# Autodesk Inventor assembly: GarageAndBracketFlatBracket
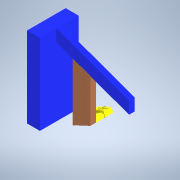
[picture p0: Inventor's stored thumbnail of the model, 180x180]
Saved by Autodesk Inventor 2022.2 (Build 262287000, 287)
## iProperties
Created: 2021-11-26
Part Number: GarageAndBracketFlatBracket
Document SubType Name: Assembly
Designer: robst
Author: robst
## Documents named in this file (4)
- C:\git\CAD-Development\robSteele\ShapeWays\GlobalMeteorNetwork\GarageAndBracketFlatBracket.iam
- C:\git\CAD-Development\robSteele\ShapeWays\GlobalMeteorNetwork\GarageSegment.ipt
- C:\git\CAD-Development\robSteele\ShapeWays\GlobalMeteorNetwork\caseLowerPortionV02.ipt
- C:\git\CAD-Development\robSteele\ShapeWays\GlobalMeteorNetwork\2x6SupportBracket.ipt
## Components (3 placed, 3 different names)
1. GarageSegment:1 — Mate:1, Mate:2, Flush:1
2. caseLowerPortionV02:1 — Flush:2, Mate:3, Mate:4
3. 2x6SupportBracket:1 — Mate:1, Mate:2, Flush:1, Flush:2, Mate:3, Mate:4
## Relationships (6: Mate 4, Flush 2)
- Mate:1: GarageSegment:1 ↔ 2x6SupportBracket:1
- Mate:2 (127 mm): GarageSegment:1 ↔ 2x6SupportBracket:1
- Flush:1: GarageSegment:1 ↔ 2x6SupportBracket:1
- Flush:2: caseLowerPortionV02:1 ↔ 2x6SupportBracket:1
- Mate:3: caseLowerPortionV02:1 ↔ 2x6SupportBracket:1
- Mate:4: caseLowerPortionV02:1 ↔ 2x6SupportBracket:1
